# Autodesk Inventor assembly: Корпус.v.2.0
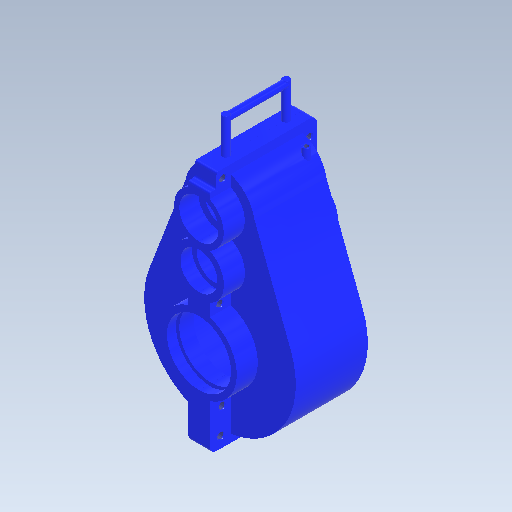
[picture p0: Inventor's stored thumbnail of the model, 512x512]
Saved by Autodesk Inventor 2021 (Build 250183000, 183)
## iProperties
Created: 2023-03-25
Part Number: Корпус.v.2.0
Document SubType Name: Assembly
Designer: gdevc
Mass: 1693.71 g
Surface Area: 4483.52 cm^2
Volume: 1693.71 cm^3
Density: 1 g/cm^3
Author: gdevc
## Documents named in this file (3)
- C:\Users\gdevc\OneDrive\Рабочий стол\Курсач\DetaliMashine\Новая папка\Корпус.v.2.0.iam
- C:\Users\gdevc\OneDrive\Рабочий стол\Курсач\DetaliMashine\Новая папка\Левая створка.ipt
- C:\Users\gdevc\OneDrive\Рабочий стол\Курсач\DetaliMashine\Новая папка\Правая створка.ipt
## Components (2 placed, 2 different names)
1. Левая створка:1 — Совмещение:1, Совмещение:2
2. Правая створка:1 — Совмещение:1, Совмещение:2
## Relationships (2: Mate 2)
- Совмещение:1 [Mate]: Левая створка:1 ↔ Правая створка:1
- Совмещение:2 [Mate]: Левая створка:1 ↔ Правая створка:1
